# Autodesk Inventor assembly: A2017_T4_08
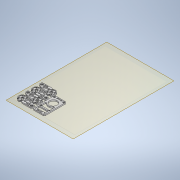
[picture p0: Inventor's stored thumbnail of the model, 180x180]
Saved by Autodesk Inventor 2020 (Build 240168000, 168)
## iProperties
Created: 2021-08-27
Part Number: A2017_T4_08
Document SubType Name: Assembly
Designer: Masato
Author: Masato
## Documents named in this file (4)
- C:\Users\naoki\Documents\Inventor\CitBrains\git_clone\SUSTAINA_ver1_0\A_T2_175\SUSTAINA-OP\Cam\A2017_T4_08.iam
- C:\Users\naoki\Documents\Inventor\CitBrains\git_clone\SUSTAINA_ver1_0\A_T2_175\SUSTAINA-OP\Cam\DisposableBoard.ipt
- C:\Users\naoki\Documents\Inventor\CitBrains\git_clone\SUSTAINA_ver1_0\A_T2_175\SUSTAINA-OP\LowerBody\Ankle\Ankle_side_pitch_frame.ipt
- C:\Users\naoki\Documents\Inventor\CitBrains\git_clone\SUSTAINA_ver1_0\A_T2_175\SUSTAINA-OP\UpperBody\Trunk\Trunk_neck_frame.ipt
## Components (6 placed, 3 different names)
1. DisposableBoard:1 — メイト:2, メイト:1, フラッシュ:1, フラッシュ:2, メイト:4, フラッシュ:3, 正接:2, メイト:5, 正接:3, メイト:7, フラッシュ:4
2. Trunk_neck_frame:1 — メイト:7, フラッシュ:4, 正接:4
3. Ankle_side_pitch_frame:1 — メイト:4, フラッシュ:3, 正接:2, メイト:6
4. Ankle_side_pitch_frame:2 — メイト:5, メイト:6, 正接:3, 正接:4
5. Ankle_side_pitch_frame:3
6. Ankle_side_pitch_frame:4
## Component patterns: (2 elements, first: Ankle_side_pitch_frame:1 + Ankle_side_pitch_frame:2)
## Relationships (13: Mate 6, Flush 4, Tangent 3)
- メイト:2 [Mate]: DisposableBoard:1
- メイト:1 [Mate]: DisposableBoard:1
- フラッシュ:1 [Flush]: DisposableBoard:1
- フラッシュ:2 [Flush]: DisposableBoard:1
- メイト:4 [Mate]: DisposableBoard:1 ↔ Ankle_side_pitch_frame:1
- フラッシュ:3 [Flush] (-2 mm): DisposableBoard:1 ↔ Ankle_side_pitch_frame:1
- 正接:2 [Tangent] (2 mm): DisposableBoard:1 ↔ Ankle_side_pitch_frame:1
- メイト:5 [Mate]: DisposableBoard:1 ↔ Ankle_side_pitch_frame:2
- メイト:6 [Mate] (2.5 mm): Ankle_side_pitch_frame:1 ↔ Ankle_side_pitch_frame:2
- 正接:3 [Tangent] (2 mm): DisposableBoard:1 ↔ Ankle_side_pitch_frame:2
- メイト:7 [Mate]: DisposableBoard:1 ↔ Trunk_neck_frame:1
- フラッシュ:4 [Flush] (2 mm): DisposableBoard:1 ↔ Trunk_neck_frame:1
- 正接:4 [Tangent] (2.5 mm): Trunk_neck_frame:1 ↔ Ankle_side_pitch_frame:2
